# Autodesk Inventor assembly: full deadbolt controller enclosure assembly
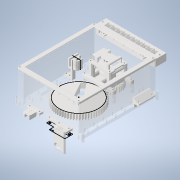
[picture p0: Inventor's stored thumbnail of the model, 180x180]
Saved by Autodesk Inventor 2022 (Build 260153000, 153)
## iProperties
Created: 2022-01-25
Part Number: full deadbolt controller enclosure assembly
Document SubType Name: Assembly
Designer: alecw
Author: alecw
## Documents named in this file (13)
- W:\My Drive\Coding and Projects\smart home\smart-deadbolt\3D Modelling\full deadbolt controller enclosure assembly.iam
- W:\My Drive\Coding and Projects\smart home\smart-deadbolt\3D Modelling\door backplate.ipt
- W:\My Drive\Coding and Projects\smart home\smart-deadbolt\3D Modelling\motor mount plate.iam
- W:\My Drive\Coding and Projects\smart home\smart-deadbolt\3D Modelling\door top plate with window.ipt
- W:\My Drive\Coding and Projects\smart home\smart-deadbolt\3D Modelling\motor gear.ipt
- W:\My Drive\Coding and Projects\smart home\smart-deadbolt\3D Modelling\motor holder top.ipt
- W:\My Drive\Coding and Projects\smart home\smart-deadbolt\3D Modelling\deadbolt enclosure walls.ipt
- W:\My Drive\Coding and Projects\smart home\smart-deadbolt\3D Modelling\limit switch mount.ipt
- W:\My Drive\Coding and Projects\smart home\smart-deadbolt\3D Modelling\ultrasonic mount to deadbolt enclosure.ipt
- W:\My Drive\Coding and Projects\smart home\smart-deadbolt\3D Modelling\led bar assembly.iam
- W:\My Drive\Coding and Projects\smart home\smart-deadbolt\3D Modelling\enclosure mounter.ipt
- W:\My Drive\Coding and Projects\smart home\smart-deadbolt\3D Modelling\deadbolt arm adapter gear straight teeth.ipt
- W:\My Drive\Coding and Projects\smart home\smart-deadbolt\3D Modelling\power and ground splitter holders.ipt
## Components (12 placed, 12 different names)
1. door backplate:1 — Flush:3, Flush:4, Mate:16, Mate:17, Mate:19, Mate:22, Mate:23, Mate:25, Mate:26, Mate:27, Mate:30, Mate:31, Mate:32, Mate:33, Mate:36, Mate:37, Mate:40, Mate:41, Mate:42, Mate:43, Rotational:1, Mate:44, Mate:45, Mate:46
2. motor mount plate:1 [sub-assembly] — Mate:11, Mate:12, Mate:13, Mate:39, Mate:40, Mate:41, Mate:42, Rotational:2
3. door top plate with window:1 — Flush:3, Flush:4, Mate:28
4. motor gear:1 — Mate:39, Rotation:1, Rotational:2
5. motor holder top:1 — Mate:11, Mate:12, Mate:13
6. deadbolt enclosure walls:1 — Mate:16, Mate:17, Mate:19, Mate:28, Flush:5, Mate:29, Mate:34, Mate:35
7. limit switch mount:1 — Mate:22, Mate:23, Mate:36
8. ultrasonic mount to deadbolt enclosure:1 — Mate:25, Mate:26, Mate:27
9. led bar assembly:1 [sub-assembly] — Flush:5, Mate:29, Mate:35
10. enclosure mounter:1 — Mate:30, Mate:31, Mate:32
11. deadbolt arm adapter gear straight teeth:1 — Mate:37, Rotation:1, Rotational:1
12. power and ground splitter holders:1 — Mate:44, Mate:45, Mate:46
## Relationships (35: Mate 29, Flush 3, RevoluteJoint 2, RelateRotation 1)
- Flush:3: door backplate:1 ↔ door top plate with window:1
- Flush:4: door backplate:1 ↔ door top plate with window:1
- Mate:11: motor mount plate:1 ↔ motor holder top:1
- Mate:12: motor mount plate:1 ↔ motor holder top:1
- Mate:13: motor mount plate:1 ↔ motor holder top:1
- Mate:16: door backplate:1 ↔ deadbolt enclosure walls:1
- Mate:17: door backplate:1 ↔ deadbolt enclosure walls:1
- Mate:19: door backplate:1 ↔ deadbolt enclosure walls:1
- Mate:22: door backplate:1 ↔ limit switch mount:1
- Mate:23: door backplate:1 ↔ limit switch mount:1
- Mate:25: door backplate:1 ↔ ultrasonic mount to deadbolt enclosure:1
- Mate:26: door backplate:1 ↔ ultrasonic mount to deadbolt enclosure:1
- Mate:27 (-3.2 mm): door backplate:1 ↔ ultrasonic mount to deadbolt enclosure:1
- Mate:28: door top plate with window:1 ↔ deadbolt enclosure walls:1
- Flush:5: deadbolt enclosure walls:1 ↔ led bar assembly:1
- Mate:29: deadbolt enclosure walls:1 ↔ led bar assembly:1
- Mate:30 (-6.4 mm): door backplate:1 ↔ enclosure mounter:1
- Mate:31 (-3.2 mm): door backplate:1 ↔ enclosure mounter:1
- Mate:32: door backplate:1 ↔ enclosure mounter:1
- Mate:33: door backplate:1
- Mate:34: deadbolt enclosure walls:1
- Mate:35: deadbolt enclosure walls:1 ↔ led bar assembly:1
- Mate:36 (-6.4 mm): door backplate:1 ↔ limit switch mount:1
- Mate:37: door backplate:1 ↔ deadbolt arm adapter gear straight teeth:1
- Mate:39: motor mount plate:1 ↔ motor gear:1
- Mate:40: door backplate:1 ↔ motor mount plate:1
- Mate:41: door backplate:1 ↔ motor mount plate:1
- Mate:42: door backplate:1 ↔ motor mount plate:1
- Mate:43: door backplate:1
- Rotation:1 [RelateRotation] (0.5 ul): motor gear:1 ↔ deadbolt arm adapter gear straight teeth:1
- Rotational:1 [RevoluteJoint] (-14 mm): door backplate:1 ↔ deadbolt arm adapter gear straight teeth:1
- Rotational:2 [RevoluteJoint] (-1 mm): motor mount plate:1 ↔ motor gear:1
- Mate:44: door backplate:1 ↔ power and ground splitter holders:1
- Mate:45: door backplate:1 ↔ power and ground splitter holders:1
- Mate:46: door backplate:1 ↔ power and ground splitter holders:1
